# Autodesk Inventor assembly: TestAssembly_02
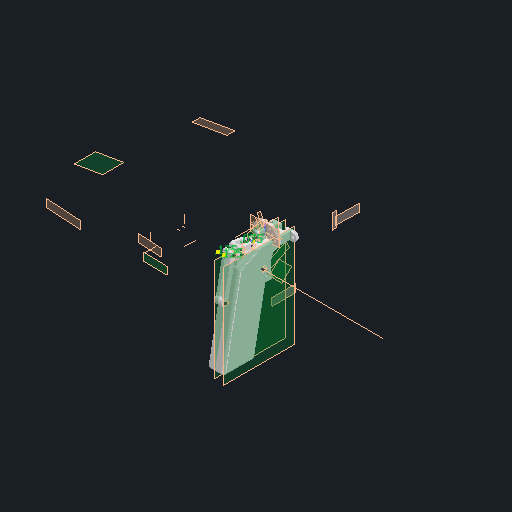
[picture p0: Inventor's stored thumbnail of the model, 512x512]
Saved by Autodesk Inventor 2024.1 (Build 281209000, 209)
## iProperties
Created: 2023-08-23
Part Number: TestAssembly_02
Document SubType Name: Assembly
Designer: Eleanor
Author: Eleanor
## Documents named in this file (14)
- C:\Users\Eleanor\Documents\Inventor\4.5mm ERS\TestAssembly_02.iam
- GripAssembly MK.001.iam
- C:\Users\Eleanor\Documents\Inventor\4.5mm ERS\SlottedHandGrip.ipt
- C:\Users\Eleanor\Documents\Inventor\4.5mm ERS\Trigger.ipt
- C:\Users\Eleanor\Documents\Inventor\4.5mm ERS\TestAssembly_02\Design Accelerator\Clevis Pin Connection1.iam
- C:\Users\Eleanor\Documents\Inventor\4.5mm ERS\LeverHolder.ipt
- C:\Users\Eleanor\Documents\Inventor\4.5mm ERS\UpperLever.ipt
- C:\Users\Eleanor\Documents\Inventor\4.5mm ERS\LowerArm.ipt
- C:\Users\Eleanor\Documents\Inventor\4.5mm ERS\WireBarrelComponent_B.iam
- C:\Users\Eleanor\Documents\Inventor\Content Center Files\R2024\en-US\ISO 7380-1\ISO 7380-1 - M3 x 12.ipt
- C:\Users\Eleanor\Documents\Inventor\4.5mm ERS\FiringPinConnectorPlate.ipt
- C:\Users\Eleanor\Documents\Inventor\4.5mm ERS\FiringPinHolder.ipt
- C:\Users\Eleanor\Documents\Inventor\4.5mm ERS\Compress Spring12.ipt
- C:\Users\Eleanor\Documents\Inventor\4.5mm ERS\TestAssembly_02\Design Accelerator\Clevis Pin Connection2.iam
## Components (18 placed, 11 different names)
1. SlottedHandGrip:1 — Mate:1, Mate:2, Mate:4, Mate:7, Mate:8, Mate:9, Flush:1, Mate:16, Angle:1, Symmetry:1, Mate:17, Mate:18
2. Trigger:1 — Mate:6, Mate:7, Mate:12, Mate:14, Mate:31
3. Clevis Pin Connection:1 [sub-assembly] — Mate:4, Mate:5, Mate:6
4. LeverHolder:1 — Mate:8, Mate:9, Flush:1, Mate:10, Mate:11, Mate:41, Mate:42
5. UpperLever:1 — Mate:10, Mate:11, Mate:13, Mate:15, Mate:19, Mate:21
6. LowerArm:1 — Mate:12, Mate:13, Mate:32, Mate:34, Mate:35, Mate:46, Mate:49
7. LowerArm:2 — Mate:14, Mate:15
8. WireBarrelComponent_B:1 [sub-assembly] — Mate:17, Mate:18, Mate:25
9. ISO 7380-1 M3 x 12:1 — Mate:25, Mate:26, Mate:29, Mate:30
10. FiringPinConnectorPlate:1 — Mate:19, Mate:20, Mate:23, Mate:28, Mate:37, Mate:38, Mate:40, Mate:44, Mate:50
11. FiringPinConnectorPlate:2 — Mate:21, Mate:28
12. FiringPinHolder:1 — Mate:20, Mate:23, Mate:26, Mate:29, Flush:2
13. Compress Spring1:1 — Mate:30, Flush:2
14. Clevis Pin Connection:2 [sub-assembly] — Mate:46, Mate:47
15. Clevis Pin Connection:3 [sub-assembly] — Mate:48
16. Clevis Pin Connection:4 [sub-assembly] — Mate:49
17. Clevis Pin Connection:5 [sub-assembly] — Mate:50
18. Clevis Pin Connection:6 [sub-assembly] — Mate:51
## Relationships (52: Mate 48, Flush 2, Angle 1, Symmetry 1)
- Mate:1: SlottedHandGrip:1
- Mate:2: SlottedHandGrip:1
- Mate:3
- Mate:4: SlottedHandGrip:1 ↔ Clevis Pin Connection:1
- Mate:5: Clevis Pin Connection:1
- Mate:6: Trigger:1 ↔ Clevis Pin Connection:1
- Mate:7: SlottedHandGrip:1 ↔ Trigger:1
- Mate:8: SlottedHandGrip:1 ↔ LeverHolder:1
- Mate:9: SlottedHandGrip:1 ↔ LeverHolder:1
- Flush:1: SlottedHandGrip:1 ↔ LeverHolder:1
- Mate:10: LeverHolder:1 ↔ UpperLever:1
- Mate:11: LeverHolder:1 ↔ UpperLever:1
- Mate:12: Trigger:1 ↔ LowerArm:1
- Mate:13: UpperLever:1 ↔ LowerArm:1
- Mate:14: Trigger:1 ↔ LowerArm:2
- Mate:15: UpperLever:1 ↔ LowerArm:2
- Mate:16: SlottedHandGrip:1
- Angle:1 (0 deg): SlottedHandGrip:1
- Symmetry:1: SlottedHandGrip:1
- Mate:17: SlottedHandGrip:1 ↔ WireBarrelComponent_B:1
- Mate:18: SlottedHandGrip:1 ↔ WireBarrelComponent_B:1
- Mate:19: UpperLever:1 ↔ FiringPinConnectorPlate:1
- Mate:20: FiringPinConnectorPlate:1 ↔ FiringPinHolder:1
- Mate:21: UpperLever:1 ↔ FiringPinConnectorPlate:2
- Mate:23: FiringPinConnectorPlate:1 ↔ FiringPinHolder:1
- Mate:25: WireBarrelComponent_B:1 ↔ ISO 7380-1 M3 x 12:1
- Mate:26: ISO 7380-1 M3 x 12:1 ↔ FiringPinHolder:1
- Mate:28: FiringPinConnectorPlate:1 ↔ FiringPinConnectorPlate:2
- Mate:29: ISO 7380-1 M3 x 12:1 ↔ FiringPinHolder:1
- Mate:30: ISO 7380-1 M3 x 12:1 ↔ Compress Spring1:1
- Flush:2: FiringPinHolder:1 ↔ Compress Spring1:1
- Mate:31: Trigger:1
- Mate:32: LowerArm:1
- Mate:33
- Mate:34: LowerArm:1
- Mate:35: LowerArm:1
- Mate:36
- Mate:37: FiringPinConnectorPlate:1
- Mate:38: FiringPinConnectorPlate:1
- Mate:39
- Mate:40: FiringPinConnectorPlate:1
- Mate:41: LeverHolder:1
- Mate:42: LeverHolder:1
- Mate:43
- Mate:44: FiringPinConnectorPlate:1
- Mate:45
- Mate:46: LowerArm:1 ↔ Clevis Pin Connection:2
- Mate:47: Clevis Pin Connection:2
- Mate:48: Clevis Pin Connection:3
- Mate:49: LowerArm:1 ↔ Clevis Pin Connection:4
- Mate:50: FiringPinConnectorPlate:1 ↔ Clevis Pin Connection:5
- Mate:51: Clevis Pin Connection:6
